# Autodesk Inventor assembly: tavcsofogo
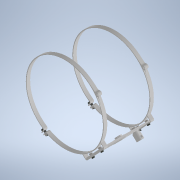
[picture p0: Inventor's stored thumbnail of the model, 180x180]
Saved by Autodesk Inventor 2021.4 (Build 254397000, 397)
## iProperties
Created: 2023-12-02
Part Number: tavcsofogo
Document SubType Name: Assembly
Designer: vtoth
Author: vtoth
## Documents named in this file (13)
- C:\Users\vtoth\OneDrive - Budapesti Műszaki és Gazdaságtudományi Egyetem\5_felev\CAD\hf2_v2\tavcsofogo.iam
- C:\Users\vtoth\OneDrive - Budapesti Műszaki és Gazdaságtudományi Egyetem\5_felev\CAD\hf2_v2\tavcso alatet.ipt
- C:\Users\vtoth\OneDrive - Budapesti Műszaki és Gazdaságtudományi Egyetem\5_felev\CAD\hf2_v2\merevito.ipt
- C:\Users\vtoth\OneDrive - Budapesti Műszaki és Gazdaságtudományi Egyetem\5_felev\CAD\hf2_v2\allemez.ipt
- C:\Users\vtoth\OneDrive - Budapesti Műszaki és Gazdaságtudományi Egyetem\5_felev\CAD\hf2_v2\tavcso csapagy.ipt
- C:\Users\vtoth\OneDrive - Budapesti Műszaki és Gazdaságtudományi Egyetem\5_felev\CAD\hf2_v2\gyuru also.ipt
- C:\Users\vtoth\OneDrive - Budapesti Műszaki és Gazdaságtudományi Egyetem\5_felev\CAD\hf2_v2\gyuru felso.ipt
- C:\Users\vtoth\OneDrive - Budapesti Műszaki és Gazdaságtudományi Egyetem\5_felev\CAD\hf2_v2\zsaner szegecs.ipt
- C:\Users\vtoth\OneDrive - Budapesti Műszaki és Gazdaságtudományi Egyetem\5_felev\CAD\hf2_v2\tavcso anya.ipt
- C:\Users\vtoth\OneDrive - Budapesti Műszaki és Gazdaságtudományi Egyetem\5_felev\CAD\hf2_v2\ContentCenter\en-US\ISO 4018\ISO 4018 - M6 x 12.ipt
- C:\Users\vtoth\OneDrive - Budapesti Műszaki és Gazdaságtudományi Egyetem\5_felev\CAD\hf2_v2\ContentCenter\en-US\ISO 4018\ISO 4018 - M8 x 20.ipt
- C:\Users\vtoth\OneDrive - Budapesti Műszaki és Gazdaságtudományi Egyetem\5_felev\CAD\hf2_v2\ContentCenter\en-US\ISO 4032(2)\ISO 4032 - M8 - ISO.ipt
- C:\Users\vtoth\OneDrive - Budapesti Műszaki és Gazdaságtudományi Egyetem\5_felev\CAD\hf2_v2\ContentCenter\en-US\ISO 4032(2)\ISO 4032 - M6 - ISO.ipt
## Components (21 placed, 12 different names)
1. tavcso alatet:1 — Insert:1
2. merevito:1 — Insert:1, Insert:2
3. allemez:1 — Insert:2, Insert:3, Insert:4, Mate:1, Mate:2, Mate:3, Insert:15, Insert:16, Insert:17, Insert:18, Insert:19
4. tavcso csapagy:1 — Insert:4
5. gyuru also:1 — Insert:6, Mate:1, Mate:2, Mate:3, Insert:7, Insert:8, Insert:9, Insert:10, Insert:13, Insert:14
6. gyuru felso:1 — Insert:5, Insert:6, Insert:11, Insert:12
7. zsaner szegecs:1 — Insert:5
8. tavcso anya:1 — Insert:3
9. ISO 4018 M6 x 12:1 — Insert:7
10. ISO 4018 M6 x 12:2 — Insert:8
11. ISO 4018 M6 x 12:3 — Insert:9
12. ISO 4018 M6 x 12:4 — Insert:10
13. ISO 4018 M8 x 20:1 — Insert:12, Mate:4
14. ISO 4018 M8 x 20:2 — Insert:11
15. ISO 4032 M8:1 — Insert:13, Mate:4
16. ISO 4032 M8:2 — Insert:14
17. ISO 4032 M6:1 — Insert:17
18. ISO 4032 M6:2 — Insert:18
19. ISO 4032 M6:3 — Insert:15
20. ISO 4032 M6:4 — Insert:16
21. ISO 4032 M8:3 — Insert:19
## Relationships (23: Insert 19, Mate 4)
- Insert:1: tavcso alatet:1 ↔ merevito:1
- Insert:2: merevito:1 ↔ allemez:1
- Insert:3: allemez:1 ↔ tavcso anya:1
- Insert:4: allemez:1 ↔ tavcso csapagy:1
- Insert:5: gyuru felso:1 ↔ zsaner szegecs:1
- Insert:6: gyuru also:1 ↔ gyuru felso:1
- Mate:1: allemez:1 ↔ gyuru also:1
- Mate:2: allemez:1 ↔ gyuru also:1
- Mate:3: allemez:1 ↔ gyuru also:1
- Insert:7: gyuru also:1 ↔ ISO 4018 M6 x 12:1
- Insert:8: gyuru also:1 ↔ ISO 4018 M6 x 12:2
- Insert:9: gyuru also:1 ↔ ISO 4018 M6 x 12:3
- Insert:10: gyuru also:1 ↔ ISO 4018 M6 x 12:4
- Insert:11: gyuru felso:1 ↔ ISO 4018 M8 x 20:2
- Insert:12: gyuru felso:1 ↔ ISO 4018 M8 x 20:1
- Insert:13: gyuru also:1 ↔ ISO 4032 M8:1
- Insert:14: gyuru also:1 ↔ ISO 4032 M8:2
- Insert:15: allemez:1 ↔ ISO 4032 M6:3
- Insert:16: allemez:1 ↔ ISO 4032 M6:4
- Insert:17: allemez:1 ↔ ISO 4032 M6:1
- Insert:18: allemez:1 ↔ ISO 4032 M6:2
- Insert:19: allemez:1 ↔ ISO 4032 M8:3
- Mate:4: ISO 4018 M8 x 20:1 ↔ ISO 4032 M8:1
